# Autodesk Inventor assembly: UpperBody
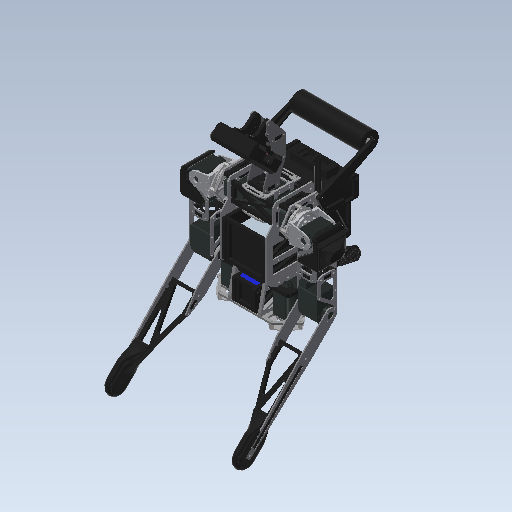
[picture p0: Inventor's stored thumbnail of the model, 512x512]
Saved by Autodesk Inventor 2020.4 (Build 244396000, 396)
## iProperties
Created: 2016-05-03
Part Number: UpperBody
Document SubType Name: Assembly
Designer: hiroaki
Mass: 2418.75 g
Surface Area: 7999.73 cm^2
Volume: 1434.4 cm^3
Density: 1.68624 g/cm^3
Author: hiroaki
## Documents named in this file (7)
- C:\Users\masato\Desktop\OpenPlatform_ver3_0\UpperBody.iam
- C:\Users\masato\Desktop\OpenPlatform_ver3_0\UpperBody\Trunk\Trunk.iam
- C:\Users\masato\Desktop\OpenPlatform_ver3_0\UpperBody\Head\Head.iam
- C:\Users\masato\Desktop\OpenPlatform_ver3_0\UpperBody\Arm\ForeArm.iam
- C:\Users\masato\Desktop\OpenPlatform_ver3_0\UpperBody\Arm\Shoulder.iam
- C:\Users\masato\Desktop\OpenPlatform_ver3_0\UpperBody\Arm\UpperArm.iam
- C:\Users\masato\Desktop\OpenPlatform_ver3_0\UpperBody\Arm\SideBumper.ipt
## Components (10 placed, 6 different names)
1. Head:1 [sub-assembly] — 挿入:13, 角度:12
2. Trunk:1 [sub-assembly] — 挿入:13, 角度:12, 挿入:14, 挿入:17, 角度:13, 角度:14
3. ForeArm:1 [sub-assembly] — 角度:18, 挿入:21, 角度:19
4. Shoulder:1 [sub-assembly] — 挿入:14, 角度:13, 挿入:20
5. UpperArm:1 [sub-assembly] — 挿入:20, 挿入:21, 角度:19, メイト:4, 角度:20, メイト:5
6. ForeArm:2 [sub-assembly] — 挿入:19, 角度:18
7. Shoulder:2 [sub-assembly] — 挿入:17, 挿入:18, 角度:14, 角度:16
8. UpperArm:2 [sub-assembly] — 挿入:18, 挿入:19, 角度:16, メイト:3, 角度:21, メイト:6
9. SideBumper:1 — メイト:4, 角度:20, メイト:5
10. SideBumper:2 — メイト:3, 角度:21, メイト:6
## Relationships (19: Angle 8, Insert 7, Mate 4)
- 挿入:13 [Insert]: Head:1 ↔ Trunk:1
- 角度:12 [Angle] (0 deg): Head:1 ↔ Trunk:1
- 挿入:14 [Insert]: Trunk:1 ↔ Shoulder:1
- 挿入:17 [Insert]: Trunk:1 ↔ Shoulder:2
- 挿入:18 [Insert]: Shoulder:2 ↔ UpperArm:2
- 挿入:19 [Insert]: ForeArm:2 ↔ UpperArm:2
- 角度:13 [Angle] (0 deg): Trunk:1 ↔ Shoulder:1
- 角度:14 [Angle] (0 deg): Trunk:1 ↔ Shoulder:2
- 角度:16 [Angle] (90 deg): Shoulder:2 ↔ UpperArm:2
- 角度:18 [Angle] (0 deg): ForeArm:1 ↔ ForeArm:2
- 挿入:20 [Insert]: Shoulder:1 ↔ UpperArm:1
- 挿入:21 [Insert]: ForeArm:1 ↔ UpperArm:1
- 角度:19 [Angle] (45 deg): ForeArm:1 ↔ UpperArm:1
- メイト:3 [Mate]: UpperArm:2 ↔ SideBumper:2
- メイト:4 [Mate]: UpperArm:1 ↔ SideBumper:1
- 角度:20 [Angle] (0 deg): UpperArm:1 ↔ SideBumper:1
- メイト:5 [Mate]: UpperArm:1 ↔ SideBumper:1
- 角度:21 [Angle] (0 deg): UpperArm:2 ↔ SideBumper:2
- メイト:6 [Mate]: UpperArm:2 ↔ SideBumper:2
